# Autodesk Inventor assembly: Chamber Top Assembly
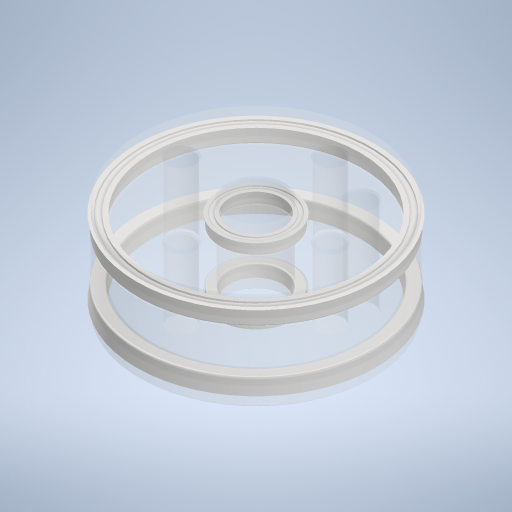
[picture p0: Inventor's stored thumbnail of the model, 512x512]
Saved by Autodesk Inventor 2024 (Build 280153000, 153)
## iProperties
Created: 2024-04-17
Part Number: Chamber Top Assembly
Document SubType Name: Assembly
Designer: Tommy Rohmann
Author: Tommy Rohmann
## Documents named in this file (4)
- C:\Users\Tommy Rohmann\Documents\Repositories\Microgravity-Press-Washing-Machine\Sub-System Design and Documentation\2 Chamber Top Assembly\Chamber Top Assembly.iam
- C:\Users\Tommy Rohmann\Documents\Repositories\Microgravity-Press-Washing-Machine\Sub-System Design and Documentation\2 Chamber Top Assembly\1 Piston Seal 4 OD O-Ring-Loaded U-Cup Seal.ipt
- C:\Users\Tommy Rohmann\Documents\Repositories\Microgravity-Press-Washing-Machine\Sub-System Design and Documentation\2 Chamber Top Assembly\2 Shaft Seal 0.875 ID O-Ring-Loaded U-Cup Seal.ipt
- C:\Users\Tommy Rohmann\Documents\Repositories\Microgravity-Press-Washing-Machine\Sub-System Design and Documentation\2 Chamber Top Assembly\3 Chamber Top Piston.ipt
## Components (5 placed, 3 different names)
1. 1 Piston Seal 4 OD O-Ring-Loaded U-Cup Seal:1 — Mate:3, Mate:4
2. 2 Shaft Seal 0.875 ID O-Ring-Loaded U-Cup Seal:1 — Mate:7, Mate:8
3. 3 Chamber Top Piston:1 — Mate:1, Mate:2, Mate:3, Mate:4, Mate:5, Mate:6, Mate:7, Mate:8
4. 1 Piston Seal 4 OD O-Ring-Loaded U-Cup Seal:2 — Mate:1, Mate:2
5. 2 Shaft Seal 0.875 ID O-Ring-Loaded U-Cup Seal:2 — Mate:5, Mate:6
## Relationships (8: Mate 8)
- Mate:1: 3 Chamber Top Piston:1 ↔ 1 Piston Seal 4 OD O-Ring-Loaded U-Cup Seal:2
- Mate:2: 3 Chamber Top Piston:1 ↔ 1 Piston Seal 4 OD O-Ring-Loaded U-Cup Seal:2
- Mate:3: 1 Piston Seal 4 OD O-Ring-Loaded U-Cup Seal:1 ↔ 3 Chamber Top Piston:1
- Mate:4: 1 Piston Seal 4 OD O-Ring-Loaded U-Cup Seal:1 ↔ 3 Chamber Top Piston:1
- Mate:5: 3 Chamber Top Piston:1 ↔ 2 Shaft Seal 0.875 ID O-Ring-Loaded U-Cup Seal:2
- Mate:6: 3 Chamber Top Piston:1 ↔ 2 Shaft Seal 0.875 ID O-Ring-Loaded U-Cup Seal:2
- Mate:7: 2 Shaft Seal 0.875 ID O-Ring-Loaded U-Cup Seal:1 ↔ 3 Chamber Top Piston:1
- Mate:8: 2 Shaft Seal 0.875 ID O-Ring-Loaded U-Cup Seal:1 ↔ 3 Chamber Top Piston:1
